# Autodesk Inventor assembly: Arm for Gen 2
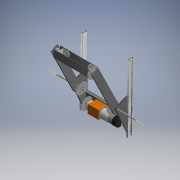
[picture p0: Inventor's stored thumbnail of the model, 180x180]
Saved by Autodesk Inventor 2019 (Build 230136000, 136)
## iProperties
Part Number: Arm for Gen 2
Document SubType Name: Assembly
Designer: Delta
Author: Delta
## Documents named in this file (14)
- C:\Robotics\2019-20_CAD\Collection\Arm for Gen 2.iam
- C:\Robotics\2019-20_CAD\Collection\12 Inch Hex Axle.ipt
- C:\Robotics\COTSParts\Sprockets - AndyMark\615106.ipt
- C:\Robotics\2019-20_CAD\Collection\bar arms.ipt
- C:\Robotics\2019-20_CAD\Collection\Claw holding bars.ipt
- C:\Robotics\COTSParts\Tetrix\39270_txm-insidecconnectors.ipt
- C:\Robotics\COTSParts\Actobotics\545 parts\545364 assembly.ipt
- C:\Robotics\COTSParts\Actobotics\545 parts\545456PatternAdapter.77in.625in.ipt
- C:\Robotics\2019-20_CAD\Collection\Spacer .25D .375H.ipt
- C:\Robotics\2019-20_CAD\Collection\Wing Left.iam
- C:\Robotics\2019-20_CAD\Collection\Wing Right.iam
- C:\Robotics\2019-20_CAD\Collection\Motor mount bar.ipt
- C:\Robotics\COTSParts\Motors\am-3643 NeveRest Sport, 104-1 with Motor.ipt
- C:\Robotics\2019-20_CAD\Collection\Motor spacer.ipt
## Components (20 placed, 13 different names)
1. 12 Inch Hex Axle:1 — Mate:5, Mate:6, Mate:8, Mate:55, Mate:59, Mate:61, Mate:74
2. 615106:1 — Mate:5, Mate:51
3. bar arms:1 — Mate:6, Flush:5, Mate:41, Mate:50, Mate:75, Mate:78
4. bar arms:2 — Mate:8, Flush:5, Mate:45, Mate:51, Mate:54, Mate:77
5. Claw holding bars:1 — Mate:22, Mate:24, Mate:25, Mate:26, Angle:2, Mate:75, Mate:76
6. 615106:2 — Mate:46, Mate:47, Mate:48, Mate:49, Mate:76
7. 39270_txm-insidecconnectors:1 — Mate:25, Mate:26, Mate:31, Mate:32
8. 39270_txm-insidecconnectors:2 — Mate:22, Mate:24, Mate:29, Mate:42, Mate:43
9. 545364 assembly:1 — Mate:33, Mate:35, Mate:45, Mate:47
10. 545364 assembly:2 — Mate:37, Mate:38, Mate:39, Mate:41, Mate:50
11. 545456PatternAdapter.77in.625in:1 — Mate:31, Mate:32, Mate:33, Mate:35, Mate:46, Mate:48, Mate:49
12. 545456PatternAdapter.77in.625in:2 — Mate:29, Mate:37, Mate:38, Mate:39, Mate:42, Mate:43
13. Spacer .25D .375H:1 — Mate:54, Mate:55
14. Wing Left:1 [sub-assembly] — Mate:61, Angle:1, Angle:2, Mate:65, Mate:78
15. Wing Right:1 [sub-assembly] — Mate:59, Angle:1, Mate:63, Mate:64, Mate:77
16. Motor mount bar:1 — Mate:63, Mate:64, Mate:65, Flush:8, Mate:70, Mate:79
17. am-3643 NeveRest Sport, 104-1 with Motor:1 — Flush:6, Flush:7, Mate:72, Mate:73
18. Motor spacer:1 — Flush:6, Flush:7, Flush:8, Mate:70, Mate:73, Mate:79
19. 615106:3 — Mate:72, Flush:9
20. 615106:4 — Mate:74, Flush:9
## Relationships (48: Mate 41, Flush 5, Angle 2)
- Mate:5: 12 Inch Hex Axle:1 ↔ 615106:1
- Mate:6: 12 Inch Hex Axle:1 ↔ bar arms:1
- Mate:8: 12 Inch Hex Axle:1 ↔ bar arms:2
- Flush:5: bar arms:1 ↔ bar arms:2
- Mate:22: Claw holding bars:1 ↔ 39270_txm-insidecconnectors:2
- Mate:24: Claw holding bars:1 ↔ 39270_txm-insidecconnectors:2
- Mate:25: Claw holding bars:1 ↔ 39270_txm-insidecconnectors:1
- Mate:26: Claw holding bars:1 ↔ 39270_txm-insidecconnectors:1
- Mate:29: 39270_txm-insidecconnectors:2 ↔ 545456PatternAdapter.77in.625in:2
- Mate:31: 39270_txm-insidecconnectors:1 ↔ 545456PatternAdapter.77in.625in:1
- Mate:32: 39270_txm-insidecconnectors:1 ↔ 545456PatternAdapter.77in.625in:1
- Mate:33: 545364 assembly:1 ↔ 545456PatternAdapter.77in.625in:1
- Mate:35: 545364 assembly:1 ↔ 545456PatternAdapter.77in.625in:1
- Mate:37: 545364 assembly:2 ↔ 545456PatternAdapter.77in.625in:2
- Mate:38: 545364 assembly:2 ↔ 545456PatternAdapter.77in.625in:2
- Mate:39: 545364 assembly:2 ↔ 545456PatternAdapter.77in.625in:2
- Mate:41: bar arms:1 ↔ 545364 assembly:2
- Mate:42: 39270_txm-insidecconnectors:2 ↔ 545456PatternAdapter.77in.625in:2
- Mate:43 (0.0762 mm): 39270_txm-insidecconnectors:2 ↔ 545456PatternAdapter.77in.625in:2
- Mate:45: bar arms:2 ↔ 545364 assembly:1
- Mate:46: 615106:2 ↔ 545456PatternAdapter.77in.625in:1
- Mate:47: 615106:2 ↔ 545364 assembly:1
- Mate:48: 615106:2 ↔ 545456PatternAdapter.77in.625in:1
- Mate:49: 615106:2 ↔ 545456PatternAdapter.77in.625in:1
- Mate:50: bar arms:1 ↔ 545364 assembly:2
- Mate:51 (9.6266 mm): 615106:1 ↔ bar arms:2
- Mate:54: bar arms:2 ↔ Spacer .25D .375H:1
- Mate:55: 12 Inch Hex Axle:1 ↔ Spacer .25D .375H:1
- Mate:59: 12 Inch Hex Axle:1 ↔ Wing Right:1
- Mate:61: 12 Inch Hex Axle:1 ↔ Wing Left:1
- Angle:1 (0 deg): Wing Left:1 ↔ Wing Right:1
- Angle:2 (0 deg): Claw holding bars:1 ↔ Wing Left:1
- Mate:63: Wing Right:1 ↔ Motor mount bar:1
- Mate:64: Wing Right:1 ↔ Motor mount bar:1
- Mate:65: Wing Left:1 ↔ Motor mount bar:1
- Flush:6: am-3643 NeveRest Sport, 104-1 with Motor:1 ↔ Motor spacer:1
- Flush:7: am-3643 NeveRest Sport, 104-1 with Motor:1 ↔ Motor spacer:1
- Flush:8: Motor mount bar:1 ↔ Motor spacer:1
- Mate:70: Motor mount bar:1 ↔ Motor spacer:1
- Mate:72: am-3643 NeveRest Sport, 104-1 with Motor:1 ↔ 615106:3
- Mate:73: am-3643 NeveRest Sport, 104-1 with Motor:1 ↔ Motor spacer:1
- Mate:74: 12 Inch Hex Axle:1 ↔ 615106:4
- Flush:9: 615106:3 ↔ 615106:4
- Mate:75 (1.27 mm): bar arms:1 ↔ Claw holding bars:1
- Mate:76 (1.27 mm): Claw holding bars:1 ↔ 615106:2
- Mate:77 (1.27 mm): bar arms:2 ↔ Wing Right:1
- Mate:78 (1.27 mm): bar arms:1 ↔ Wing Left:1
- Mate:79: Motor mount bar:1 ↔ Motor spacer:1
